# Autodesk Inventor assembly: entireRobot
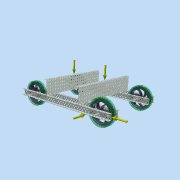
[picture p0: Inventor's stored thumbnail of the model, 180x180]
Saved by Autodesk Inventor 2015 (Build 190159000, 159)
## iProperties
Created: 2017-06-02
Part Number: entireRobot
Document SubType Name: Assembly
Designer: Tommy
Author: Tommy
## Documents named in this file (9)
- C:\Users\Tommy\Documents\GitHub\VEX-Robotics-2017-2018\Robot\entireRobot.iam
- C:\Users\Tommy\Documents\GitHub\VEX-Robotics-2017-2018\Imperial\Structure\C-Channel 1x5x1x35 Hole.iam
- C:\Users\Tommy\Documents\GitHub\VEX-Robotics-2017-2018\Imperial\Structure\C-Channel 1x5x1x25 Hole.ipt
- C:\Users\Tommy\Documents\GitHub\VEX-Robotics-2017-2018\Imperial\Motion\4 inch Wheel.iam
- C:\Users\Tommy\Documents\GitHub\VEX-Robotics-2017-2018\Imperial\Motion\Shaft 4 inch.ipt
- C:\Users\Tommy\Documents\GitHub\VEX-Robotics-2017-2018\Robot\entireRobot\AIP\FEA\c60eafb40.fins
- C:\Users\Tommy\Documents\GitHub\VEX-Robotics-2017-2018\Robot\entireRobot\AIP\FEA\c60eafcg0.fsat
- C:\Users\Tommy\Documents\GitHub\VEX-Robotics-2017-2018\Robot\entireRobot\AIP\FEA\c60eafckg.ftes
- C:\Users\Tommy\Documents\GitHub\VEX-Robotics-2017-2018\Robot\entireRobot\AIP\FEA\c60eafckg.fwiz
## Components (14 placed, 4 different names)
1. C-Channel 1x5x1x35 Hole:1 [sub-assembly] — Mate:1, Flush:1, Flush:2, Flush:3
2. C-Channel 1x5x1x35 Hole:2 [sub-assembly] — Mate:2, Flush:2, Flush:5, Flush:8, Flush:9, Insert:1, Insert:3
3. C-Channel 1x5x1x35 Hole:6 [sub-assembly] — Mate:5, Flush:6, Flush:7, Insert:2, Insert:4
4. C-Channel 1x5x1x35 Hole:7 [sub-assembly] — Mate:4, Flush:4, Flush:5, Flush:6, Mate:6
5. C-Channel 1x5x1x25 Hole:1 — Mate:1, Flush:1, Mate:2, Flush:3, Mate:4, Flush:4, Mate:5, Flush:7, Flush:8, Flush:10
6. C-Channel 1x5x1x25 Hole:2 — Mate:6, Flush:9, Flush:10
7. 4 inch Wheel:1 [sub-assembly] — Insert:1, Insert:7
8. 4 inch Wheel:2 [sub-assembly] — Insert:2, Insert:5
9. 4 inch Wheel:3 [sub-assembly] — Insert:3, Insert:8
10. 4 inch Wheel:4 [sub-assembly] — Insert:4, Insert:6
11. Shaft 4 inch:1 — Insert:7
12. Shaft 4 inch:2 — Insert:6
13. Shaft 4 inch:3 — Insert:8
14. Shaft 4 inch:4 — Insert:5
## Relationships (23: Flush 10, Insert 8, Mate 5)
- Mate:1: C-Channel 1x5x1x35 Hole:1 ↔ C-Channel 1x5x1x25 Hole:1
- Flush:1: C-Channel 1x5x1x35 Hole:1 ↔ C-Channel 1x5x1x25 Hole:1
- Mate:2: C-Channel 1x5x1x35 Hole:2 ↔ C-Channel 1x5x1x25 Hole:1
- Flush:2: C-Channel 1x5x1x35 Hole:1 ↔ C-Channel 1x5x1x35 Hole:2
- Flush:3: C-Channel 1x5x1x35 Hole:1 ↔ C-Channel 1x5x1x25 Hole:1
- Mate:4: C-Channel 1x5x1x35 Hole:7 ↔ C-Channel 1x5x1x25 Hole:1
- Flush:4: C-Channel 1x5x1x35 Hole:7 ↔ C-Channel 1x5x1x25 Hole:1
- Flush:5: C-Channel 1x5x1x35 Hole:2 ↔ C-Channel 1x5x1x35 Hole:7
- Mate:5: C-Channel 1x5x1x35 Hole:6 ↔ C-Channel 1x5x1x25 Hole:1
- Flush:6: C-Channel 1x5x1x35 Hole:6 ↔ C-Channel 1x5x1x35 Hole:7
- Flush:7: C-Channel 1x5x1x35 Hole:6 ↔ C-Channel 1x5x1x25 Hole:1
- Flush:8: C-Channel 1x5x1x35 Hole:2 ↔ C-Channel 1x5x1x25 Hole:1
- Mate:6: C-Channel 1x5x1x35 Hole:7 ↔ C-Channel 1x5x1x25 Hole:2
- Flush:9: C-Channel 1x5x1x35 Hole:2 ↔ C-Channel 1x5x1x25 Hole:2
- Flush:10: C-Channel 1x5x1x25 Hole:1 ↔ C-Channel 1x5x1x25 Hole:2
- Insert:1 (6.35 mm): C-Channel 1x5x1x35 Hole:2 ↔ 4 inch Wheel:1
- Insert:2 (6.35 mm): C-Channel 1x5x1x35 Hole:6 ↔ 4 inch Wheel:2
- Insert:3 (6.35 mm): C-Channel 1x5x1x35 Hole:2 ↔ 4 inch Wheel:3
- Insert:4 (6.35 mm): C-Channel 1x5x1x35 Hole:6 ↔ 4 inch Wheel:4
- Insert:5 (-63.5 mm): 4 inch Wheel:2 ↔ Shaft 4 inch:4
- Insert:6 (-63.5 mm): 4 inch Wheel:4 ↔ Shaft 4 inch:2
- Insert:7 (-63.5 mm): 4 inch Wheel:1 ↔ Shaft 4 inch:1
- Insert:8 (-63.5 mm): 4 inch Wheel:3 ↔ Shaft 4 inch:3
## Named parameters: sa_0 = 193.386, sa_1 = 9.34127e-12, sa_2 = -2215.69, sa_3 = -4.44822e-13, sa_4 = 5560.28, sa_5 = 1.2455e-11, sa_6 = -3545.1, sa_7 = -1.77929e-12, sa_8 = -309.418
note: some values were not read from the file. Shown as the stored number, unit unknown: "sa_0", "sa_1", "sa_2", "sa_3", "sa_4", "sa_5", "sa_6", "sa_7", "sa_8".
